# Autodesk Inventor assembly: new spool
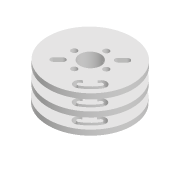
[picture p0: Inventor's stored thumbnail of the model, 180x180]
Saved by Autodesk Inventor 2020 (Build 240168000, 168)
## iProperties
Created: 2019-12-26
Part Number: new spool
Document SubType Name: Assembly
Designer: ball
Author: ball
## Documents named in this file (4)
- C:\FTC\FTC8863CAD\2019 Robot\Delivery\new spool.iam
- C:\FTC\FTC8863CAD\Actobotics\615 parts\615468 inner plate.ipt
- C:\FTC\FTC8863CAD\Actobotics\615 parts\615468 outer plate 2_0 diameter.ipt
- C:\FTC\FTC8863CAD\Actobotics\545 parts\545619 assembly.ipt
## Components (8 placed, 3 different names)
1. 615468 inner plate:1
2. 615468 outer plate 2_0 diameter:1
3. 615468 inner plate:2
4. 615468 outer plate 2_0 diameter:2
5. 615468 inner plate:3
6. 615468 inner plate:4
7. 615468 outer plate 2_0 diameter:3
8. 545619 assembly:1
## Relationships (14: Mate 14)
- [Mate]: 615468 inner plate:1 ↔ 615468 inner plate:2
- [Mate]: 615468 inner plate:1 ↔ 615468 inner plate:2
- [Mate]: 615468 inner plate:1 ↔ 615468 outer plate 2_0 diameter:1
- [Mate]: 615468 inner plate:1 ↔ 615468 outer plate 2_0 diameter:1
- [Mate]: 615468 inner plate:2 ↔ 615468 outer plate 2_0 diameter:2
- [Mate]: 615468 inner plate:2 ↔ 615468 outer plate 2_0 diameter:2
- [Mate]: 615468 inner plate:3 ↔ 615468 inner plate:4
- [Mate]: 615468 inner plate:3 ↔ 615468 inner plate:4
- [Mate]: 615468 outer plate 2_0 diameter:1 ↔ 615468 inner plate:3
- [Mate]: 615468 outer plate 2_0 diameter:1 ↔ 615468 inner plate:4
- [Mate]: 615468 inner plate:3 ↔ 615468 outer plate 2_0 diameter:3
- [Mate]: 615468 inner plate:3 ↔ 615468 outer plate 2_0 diameter:3
- [Mate]: 615468 outer plate 2_0 diameter:3 ↔ 545619 assembly:1
- [Mate]: 615468 outer plate 2_0 diameter:3 ↔ 545619 assembly:1
